# Autodesk Inventor assembly: StirnradUNDServo_MIR1
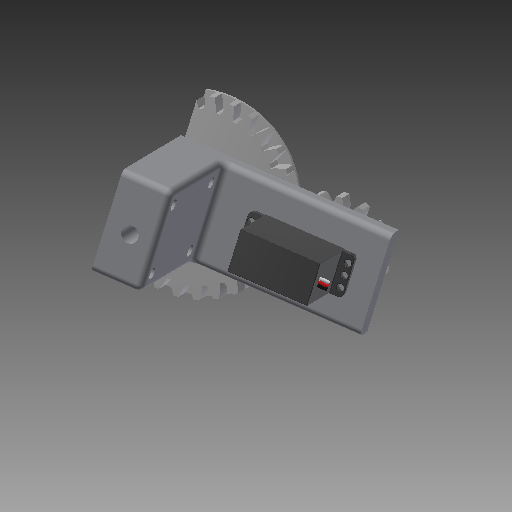
[picture p0: Inventor's stored thumbnail of the model, 512x512]
Saved by Autodesk Inventor 2018 (Build 220112000, 112)
## iProperties
Created: 2018-01-26
Part Number: StirnradUNDServo_MIR1
Material: Generisch
Document SubType Name: Assembly
Designer: gchri
Mass: 191.612 g
Surface Area: 210.73 cm^2
Volume: 54.9428 cm^3
Density: 3.48748 g/cm^3
Author: gchri
## Documents named in this file (4)
- C:\Users\Chris\OneDrive\Development\Mohne\03_Konstruktion\StirnradUNDServo_MIR1.iam
- C:\Users\Chris\OneDrive\Development\Mohne\03_Konstruktion\StirnradUNDServo\Konstruktions-Assistent\Stirnräder1_MIR1.iam
- C:\Users\Chris\OneDrive\Development\Mohne\03_Konstruktion\servo_SM-S2309S_MIR1.ipt
- C:\Users\Chris\OneDrive\Development\Mohne\03_Konstruktion\L-Halterung Servo_MIR2.ipt
## Components (3 placed, 3 different names)
1. Stirnräder1_MIR1:1 [sub-assembly] — Passend:5, Passend:4
2. servo_SM-S2309S_MIR1:1 — Passend:5, Passend:4, Passend:3, Passend:2, Passend:1
3. L-Halterung Servo_MIR2:1 — Passend:3, Passend:2, Passend:1
## Relationships (5: Mate 5)
- Passend:5 [Mate]: Stirnräder1_MIR1:1 ↔ servo_SM-S2309S_MIR1:1
- Passend:4 [Mate]: Stirnräder1_MIR1:1 ↔ servo_SM-S2309S_MIR1:1
- Passend:3 [Mate]: servo_SM-S2309S_MIR1:1 ↔ L-Halterung Servo_MIR2:1
- Passend:2 [Mate]: servo_SM-S2309S_MIR1:1 ↔ L-Halterung Servo_MIR2:1
- Passend:1 [Mate]: servo_SM-S2309S_MIR1:1 ↔ L-Halterung Servo_MIR2:1
